# Autodesk Inventor assembly: Lackieranlage
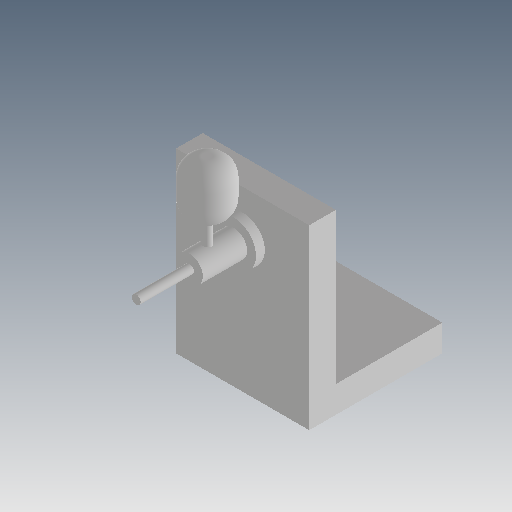
[picture p0: Inventor's stored thumbnail of the model, 512x512]
Saved by Autodesk Inventor 2020 (Build 240168000, 168)
## iProperties
Created: 2020-03-18
Part Number: Lackieranlage
Document SubType Name: Assembly
Designer: franz
Author: franz
## Documents named in this file (3)
- E:\Privat\Projekte\SPS_Training\Unity_SPS_Simulation\Unity_SPS_Schrittkette\CAD\Foerderband_V1\Lackieranlage\Lackieranlage.iam
- E:\Privat\Projekte\SPS_Training\Unity_SPS_Simulation\Unity_SPS_Schrittkette\CAD\Foerderband_V1\Lackieranlage\Staender.ipt
- E:\Privat\Projekte\SPS_Training\Unity_SPS_Simulation\Unity_SPS_Schrittkette\CAD\Foerderband_V1\Lackieranlage\Lackierkopf.ipt
## Components (2 placed, 2 different names)
1. Staender:1 — Starr:1
2. Lackierkopf:1 — Starr:1
## Relationships (1: WeldJoint 1)
- Starr:1 [WeldJoint]: Staender:1 ↔ Lackierkopf:1
